# Autodesk Inventor assembly: Tarot_12mm_Mount
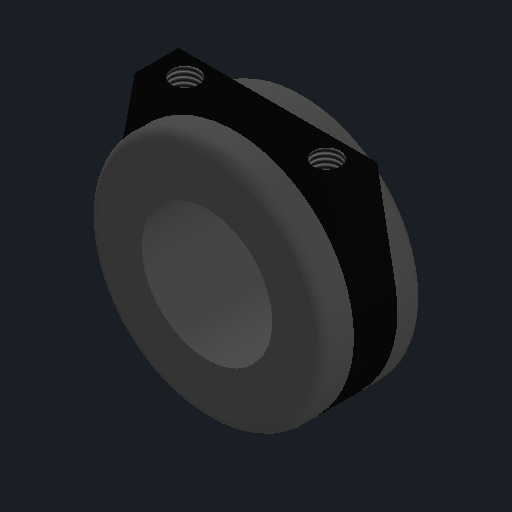
[picture p0: Inventor's stored thumbnail of the model, 512x512]
Saved by Autodesk Inventor 2024.1 (Build 281209000, 209)
## iProperties
Created: 2023-06-28
Part Number: Tarot_12mm_Mount
Document SubType Name: Assembly
Designer: dzw04
Author: dzw04
## Documents named in this file (3)
- C:\Users\dzw04\Saxion\Mechatronica Lectoraat LMECH LED - Database ARG\Component_Database\SARAX\01. CAD\01. 3D_Drawing\02. Sub_Assemblies\Miscellaneous\Tarot_12mm_Mount.iam
- C:\Users\dzw04\Saxion\Mechatronica Lectoraat LMECH LED - Database ARG\Component_Database\SARAX\01. CAD\01. 3D_Drawing\01. Parts\Tarot_12mm_Mount.ipt
- C:\Users\dzw04\Saxion\Mechatronica Lectoraat LMECH LED - Database ARG\Component_Database\SARAX\01. CAD\01. 3D_Drawing\01. Parts\Tarot_12mm_Rubber.ipt
## Components (2 placed, 2 different names)
1. Tarot_12mm_Mount:1 — Mate:1, Mate:2
2. Tarot_12mm_Rubber:1 — Mate:1, Mate:2
## Relationships (2: Mate 2)
- Mate:1: Tarot_12mm_Mount:1 ↔ Tarot_12mm_Rubber:1
- Mate:2: Tarot_12mm_Mount:1 ↔ Tarot_12mm_Rubber:1
